# Autodesk Inventor assembly: wire box and cover
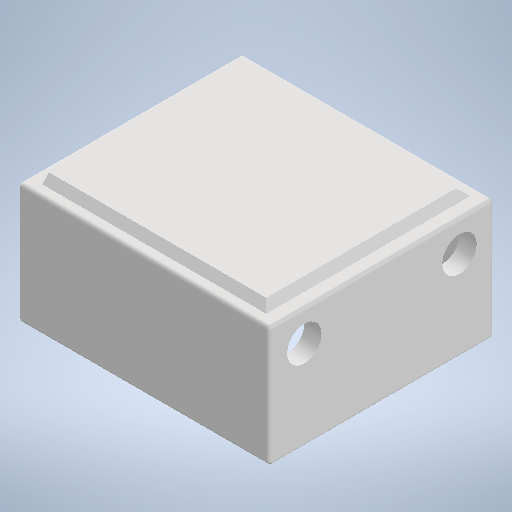
[picture p0: Inventor's stored thumbnail of the model, 512x512]
Saved by Autodesk Inventor 2025 (Build 290162000, 162)
## iProperties
Created: 2024-07-26
Part Number: wire box and cover
Document SubType Name: Assembly
Designer: Isaac
Author: Isaac
## Documents named in this file (3)
- C:\Users\Isaac\Downloads\Rack2\Rack\wire box and cover.iam
- C:\Users\Isaac\Downloads\Rack2\Rack\Part186.ipt
- C:\Users\Isaac\Downloads\Rack2\Rack\Part185.ipt
## Components (2 placed, 2 different names)
1. Part185:1 — Mate:1, Mate:2
2. Part186:1 — Mate:1, Mate:2
## Relationships (2: Mate 2)
- Mate:1: Part185:1 ↔ Part186:1
- Mate:2: Part185:1 ↔ Part186:1
